# Autodesk Inventor assembly: stepover
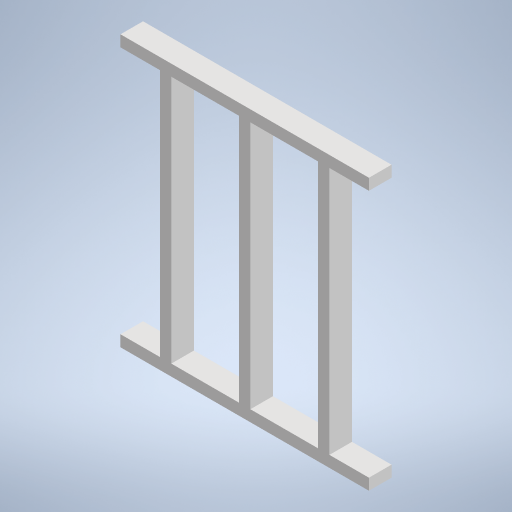
[picture p0: Inventor's stored thumbnail of the model, 512x512]
Saved by Autodesk Inventor 2024.2 (Build 282272000, 272)
## iProperties
Created: 2024-01-16
Part Number: stepover
Document SubType Name: Assembly
Designer: HukoOo
Author: HukoOo
## Documents named in this file (2)
- E:\OneDrive - 성균관대학교\Projects\2024 ICRA QRC 대회\모델\stepover.iam
- E:\OneDrive - 성균관대학교\Projects\2024 ICRA QRC 대회\모델\board_50x100x1100.ipt
## Components (5 placed, 1 different names)
1. board_50x100x1100:2 — 플러쉬:1, 플러쉬:2, 메이트:1, 메이트:2, 메이트:3, 플러쉬:3, 플러쉬:4, 플러쉬:5, 메이트:4
2. board_50x100x1100:3 — 메이트:1, 플러쉬:3, 플러쉬:7, 메이트:5
3. board_50x100x1100:4 — 메이트:2, 플러쉬:4, 메이트:5
4. board_50x100x1100:5 — 플러쉬:1, 플러쉬:2, 메이트:4, 플러쉬:6, 플러쉬:7
5. board_50x100x1100:6 — 메이트:3, 플러쉬:5, 플러쉬:6
## Relationships (12: Flush 7, Mate 5)
- 플러쉬:1 [Flush]: board_50x100x1100:2 ↔ board_50x100x1100:5
- 플러쉬:2 [Flush]: board_50x100x1100:2 ↔ board_50x100x1100:5
- 메이트:1 [Mate]: board_50x100x1100:2 ↔ board_50x100x1100:3
- 메이트:2 [Mate]: board_50x100x1100:2 ↔ board_50x100x1100:4
- 메이트:3 [Mate]: board_50x100x1100:2 ↔ board_50x100x1100:6
- 플러쉬:3 [Flush]: board_50x100x1100:2 ↔ board_50x100x1100:3
- 플러쉬:4 [Flush]: board_50x100x1100:2 ↔ board_50x100x1100:4
- 플러쉬:5 [Flush]: board_50x100x1100:2 ↔ board_50x100x1100:6
- 메이트:4 [Mate] (1100 mm): board_50x100x1100:2 ↔ board_50x100x1100:5
- 플러쉬:6 [Flush] (175 mm): board_50x100x1100:5 ↔ board_50x100x1100:6
- 플러쉬:7 [Flush] (175 mm): board_50x100x1100:3 ↔ board_50x100x1100:5
- 메이트:5 [Mate] (300 mm): board_50x100x1100:3 ↔ board_50x100x1100:4
